# Autodesk Inventor assembly: Assembly8
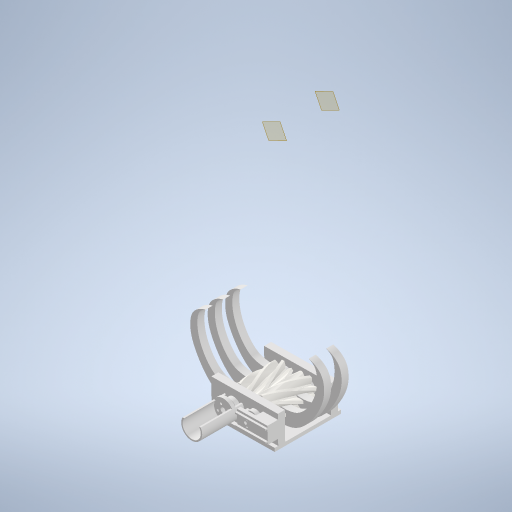
[picture p0: Inventor's stored thumbnail of the model, 512x512]
Saved by Autodesk Inventor 2023.2 (Build 272271030, 271C)
## iProperties
Created: 2023-05-17
Part Number: Assembly8
Document SubType Name: Assembly
Designer: chris
Author: chris
## Documents named in this file (5)
- C:\Users\chris\Documents\BioInsp\assembly_parts\Assembly8.iam
- C:\Users\chris\Documents\BioInsp\assembly_parts\arm_2.ipt
- C:\Users\chris\Documents\BioInsp\assembly_parts\arm_3.ipt
- C:\Users\chris\Documents\BioInsp\assembly_parts\main_base.ipt
- C:\Users\chris\Documents\BioInsp\assembly_parts\secondary_base.ipt
## Components (5 placed, 4 different names)
1. arm_2:1 — Mate:2, Flush:4
2. arm_3:1 — Mate:1, Flush:4
3. main_base:1 — Flush:1, Flush:2, Flush:3, Mate:1, Mate:2, Flush:5, Flush:6, Mate:3
4. secondary_base:1 — Flush:1, Flush:2, Flush:3
5. secondary_base:2 — Flush:5, Flush:6, Mate:3
## Relationships (9: Flush 6, Mate 3)
- Flush:1: main_base:1 ↔ secondary_base:1
- Flush:2: main_base:1 ↔ secondary_base:1
- Flush:3: main_base:1 ↔ secondary_base:1
- Mate:1: arm_3:1 ↔ main_base:1
- Mate:2: arm_2:1 ↔ main_base:1
- Flush:4: arm_2:1 ↔ arm_3:1
- Flush:5: main_base:1 ↔ secondary_base:2
- Flush:6: main_base:1 ↔ secondary_base:2
- Mate:3: main_base:1 ↔ secondary_base:2
